# Autodesk Inventor assembly: Emergency barb assembly
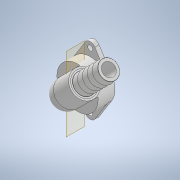
[picture p0: Inventor's stored thumbnail of the model, 180x180]
Saved by Autodesk Inventor 2020 (Build 240168000, 168)
## iProperties
Created: 2020-04-09
Part Number: Emergency barb assembly
Document SubType Name: Assembly
Designer: angusaitken
Author: angusaitken
## Documents named in this file (3)
- \\Mac\Home\Desktop\3D\Breeze thing\Breeze V2\Inlet subassembly stuff - Angus\Emergency barb assembly.iam
- \\Mac\Home\Desktop\3D\Breeze thing\Breeze V2\Inlet subassembly stuff - Angus\Emergency Barb.ipt
- \\Mac\Home\Desktop\3D\Breeze thing\Breeze V2\Inlet subassembly stuff - Angus\5346K220_BRASS BARBED HOSE FITTING.ipt
## Components (2 placed, 2 different names)
1. Emergency Barb:1 — Flush:1, Mate:1, Flush:2, Mate:2
2. 5346K220_BRASS BARBED HOSE FITTING:1 — Mate:1, Flush:2, Mate:2
## Relationships (4: Flush 2, Mate 2)
- Flush:1: Emergency Barb:1
- Mate:1: Emergency Barb:1 ↔ 5346K220_BRASS BARBED HOSE FITTING:1
- Flush:2: Emergency Barb:1 ↔ 5346K220_BRASS BARBED HOSE FITTING:1
- Mate:2: Emergency Barb:1 ↔ 5346K220_BRASS BARBED HOSE FITTING:1
